# Autodesk Inventor assembly: Shotclock
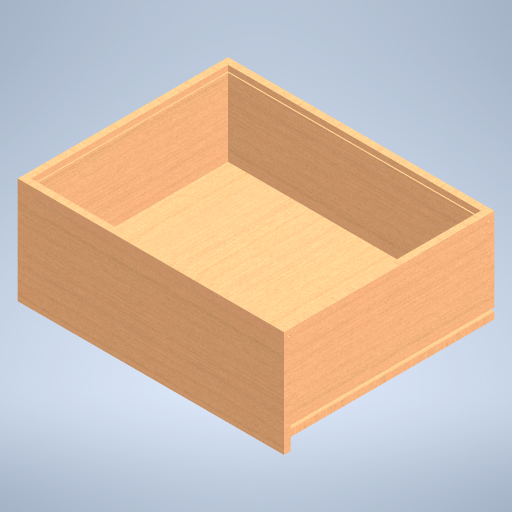
[picture p0: Inventor's stored thumbnail of the model, 512x512]
Saved by Autodesk Inventor 2024 (Build 280153000, 153)
## iProperties
Created: 2024-03-12
Part Number: Shotclock
Document SubType Name: Assembly
Designer: haniv
Author: haniv
## Documents named in this file (5)
- C:\Users\haniv\Desktop\Unterlagen\Projekte\7_Segment_Anzeige\ScoreDisplay\CAD\Shotclock.iam
- C:\Users\haniv\Desktop\Unterlagen\Projekte\7_Segment_Anzeige\ScoreDisplay\CAD\Components\Oberseite_Shotclock.ipt
- C:\Users\haniv\Desktop\Unterlagen\Projekte\7_Segment_Anzeige\ScoreDisplay\CAD\Components\Querseite_Shotclock.ipt
- C:\Users\haniv\Desktop\Unterlagen\Projekte\7_Segment_Anzeige\ScoreDisplay\CAD\Components\Unterseite_Shotclock.ipt
- C:\Users\haniv\Desktop\Unterlagen\Projekte\7_Segment_Anzeige\ScoreDisplay\CAD\Components\Rückseite_Shotclock.ipt
## Components (5 placed, 4 different names)
1. Oberseite_Shotclock:1 — Passend:1, Fluchtend:1, Fluchtend:2, Passend:2, Fluchtend:3, Fluchtend:4, Passend:4
2. Querseite_Shotclock:1 — Passend:1, Fluchtend:1, Fluchtend:2, Passend:3, Fluchtend:5, Fluchtend:7
3. Querseite_Shotclock:2 — Passend:2, Fluchtend:3, Fluchtend:4, Fluchtend:6
4. Unterseite_Shotclock:1 — Passend:3, Fluchtend:5, Fluchtend:6
5. Rückseite_Shotclock:1 — Passend:4, Fluchtend:7
## Relationships (11: Flush 7, Mate 4)
- Passend:1 [Mate]: Oberseite_Shotclock:1 ↔ Querseite_Shotclock:1
- Fluchtend:1 [Flush]: Oberseite_Shotclock:1 ↔ Querseite_Shotclock:1
- Fluchtend:2 [Flush]: Oberseite_Shotclock:1 ↔ Querseite_Shotclock:1
- Passend:2 [Mate]: Oberseite_Shotclock:1 ↔ Querseite_Shotclock:2
- Fluchtend:3 [Flush]: Oberseite_Shotclock:1 ↔ Querseite_Shotclock:2
- Fluchtend:4 [Flush]: Oberseite_Shotclock:1 ↔ Querseite_Shotclock:2
- Passend:3 [Mate]: Querseite_Shotclock:1 ↔ Unterseite_Shotclock:1
- Fluchtend:5 [Flush]: Querseite_Shotclock:1 ↔ Unterseite_Shotclock:1
- Fluchtend:6 [Flush]: Querseite_Shotclock:2 ↔ Unterseite_Shotclock:1
- Passend:4 [Mate]: Oberseite_Shotclock:1 ↔ Rückseite_Shotclock:1
- Fluchtend:7 [Flush]: Querseite_Shotclock:1 ↔ Rückseite_Shotclock:1
